# Autodesk Inventor assembly: STL Generator
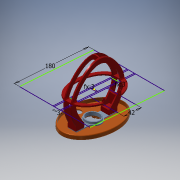
[picture p0: Inventor's stored thumbnail of the model, 180x180]
Saved by Autodesk Inventor 2018.3 (Build 223284000, 284)
## iProperties
Created: 2018-03-10
Part Number: STL Generator
Material: Generisch
Document SubType Name: Assembly
Designer: JochenAlt
Author: JochenAlt
## Documents named in this file (15)
- D:\Projects\Donna\CAD\opengl\STL Generator.iam
- D:\Projects\Donna\CAD\Donnas Head.ipt
- D:\Projects\Donna\CAD\Stewart-Base.iam
- D:\Projects\Donna\CAD\Servo-Arm-Head-20mm-Ball-Joint.iam
- D:\Projects\Donna\CAD\Stewart-Body.iam
- D:\Projects\Donna\CAD\Body-Rod.iam
- D:\Projects\Donna\CAD\Head-Rod.iam
- D:\Projects\Donna\CAD\Stewart-Head.iam
- D:\Projects\Donna\CAD\Mouth-Base.ipt
- D:\Projects\Donna\CAD\Servo-Arm-Lip.ipt
- D:\Projects\Donna\CAD\Servo-Arm-Mouth.ipt
- D:\Projects\Donna\CAD\Mouth-Height-Lever.ipt
- D:\Projects\Donna\CAD\Mouth-Height-Lever-front.ipt
- D:\Projects\Donna\CAD\Bottom-Lip.ipt
- D:\Projects\Donna\CAD\Mouth-Upper-Holder.ipt
## Components (14 placed, 12 different names)
1. Donnas Head:1 — Passend:1, Passend:2, Winkel:1
2. Stewart-Body:1 [sub-assembly] — Passend:3, Passend:4, Winkel:2
3. Servo-Arm-Head-20mm-Ball-Joint:1 [sub-assembly] — Passend:5, Passend:6, Passend:7
4. Stewart-Body [sub-assembly] — Passend:8, Passend:9, Passend:10
5. BodyRod [sub-assembly] — Passend:14, Passend:15
6. HeadRod [sub-assembly] — Passend:12, Passend:13
7. Stewart-Head:1 [sub-assembly] — Passend:16, Passend:17, Passend:41, Passend:42, Passend:43
8. Mouth-Base:1 — Passend:18, Passend:19, Winkel:3
9. ServoArm:1 — Passend:20, Passend:26
10. ServoArm:2 — Passend:22, Passend:37, Passend:39, Fluchtend:1
11. Mouth-Height-Lever:1 — Passend:30, Passend:31, Passend:32
12. LowerLip — Passend:27, Passend:29, Passend:40
13. UpperLip — Passend:33, Passend:34, Passend:35
14. Mouth-Upper-Lip-Holder:1 — Passend:41, Passend:42, Passend:43
## Relationships (39: Mate 35, Angle 3, Flush 1)
- Passend:1 [Mate]: Donnas Head:1
- Passend:2 [Mate]: Donnas Head:1
- Winkel:1 [Angle] (90 deg): Donnas Head:1
- Passend:3 [Mate]: Stewart-Body:1
- Passend:4 [Mate]: Stewart-Body:1
- Winkel:2 [Angle] (0 deg): Stewart-Body:1
- Passend:5 [Mate]: Servo-Arm-Head-20mm-Ball-Joint:1
- Passend:6 [Mate]: Servo-Arm-Head-20mm-Ball-Joint:1
- Passend:7 [Mate]: Servo-Arm-Head-20mm-Ball-Joint:1
- Passend:8 [Mate]: Stewart-Body
- Passend:9 [Mate]: Stewart-Body
- Passend:10 [Mate]: Stewart-Body
- Passend:12 [Mate]: HeadRod
- Passend:13 [Mate]: HeadRod
- Passend:14 [Mate]: BodyRod
- Passend:15 [Mate]: BodyRod
- Passend:16 [Mate]: Stewart-Head:1
- Passend:17 [Mate]: Stewart-Head:1
- Passend:18 [Mate]: Mouth-Base:1
- Passend:19 [Mate] (5 mm): Mouth-Base:1
- Winkel:3 [Angle] (90 deg): Mouth-Base:1
- Passend:20 [Mate]: ServoArm:1
- Passend:22 [Mate]: ServoArm:2
- Passend:26 [Mate]: ServoArm:1
- Passend:27 [Mate]: LowerLip
- Passend:29 [Mate] (9 mm): LowerLip
- Passend:30 [Mate]: Mouth-Height-Lever:1
- Passend:31 [Mate] (6.5 mm): Mouth-Height-Lever:1
- Passend:32 [Mate]: Mouth-Height-Lever:1
- Passend:33 [Mate]: UpperLip
- Passend:34 [Mate]: UpperLip
- Passend:35 [Mate] (17.5 mm): UpperLip
- Passend:37 [Mate] (-6 mm): ServoArm:2
- Passend:39 [Mate]: ServoArm:2
- Fluchtend:1 [Flush] (-30 mm): ServoArm:2
- Passend:40 [Mate]: LowerLip
- Passend:41 [Mate]: Stewart-Head:1 ↔ Mouth-Upper-Lip-Holder:1
- Passend:42 [Mate]: Stewart-Head:1 ↔ Mouth-Upper-Lip-Holder:1
- Passend:43 [Mate]: Stewart-Head:1 ↔ Mouth-Upper-Lip-Holder:1
